# Autodesk Inventor assembly: Assembly
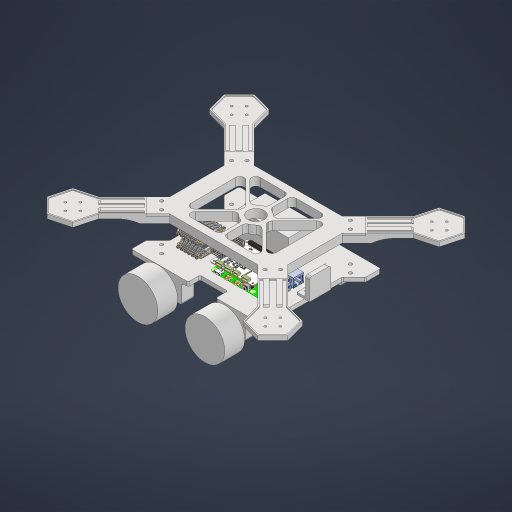
[picture p0: Inventor's stored thumbnail of the model, 512x512]
Saved by Autodesk Inventor 2023 (Build 270158000, 158)
## iProperties
Created: 2023-01-16
Part Number: Assembly
Document SubType Name: Assembly
Designer: Michael
Author: Michael
## Documents named in this file (12)
- D:\IDEs\Autodesk\SDP\Assembly.iam
- D:\IDEs\Autodesk\SDP\Base.ipt
- Electronics Panel.ipt
- D:\IDEs\Autodesk\SDP\navio2\NAVIO2.ipt
- D:\IDEs\Autodesk\SDP\raspberry-pi-4-model-b\Raspberry Pi 4 Model B.ipt
- D:\IDEs\Autodesk\SDP\tattu-4s-6750mah-lipo-battery\Tattu_4S_6750mAh_25C\Tattu_4S_6750mAh_25C.ipt
- D:\IDEs\Autodesk\SDP\LiPo.ipt
- D:\IDEs\Autodesk\SDP\ESC F45A\F45A.ipt
- D:\IDEs\Autodesk\SDP\Arm.ipt
- D:\IDEs\Autodesk\SDP\Top.ipt
- D:\IDEs\Autodesk\SDP\Camera Mount.ipt
- D:\IDEs\Autodesk\SDP\Mecanum Wheel.ipt
## Components (15 placed, 10 different names)
1. Electronics Panel:1 — Mate:25, Mate:26, Mate:33, Mate:34, Mate:35, Mate:36, Flush:5, Mate:39, Mate:40, Mate:41, Mate:42, Mate:43, Mate:44
2. NAVIO2:1 — Mate:5, Flush:1, Flush:2
3. Raspberry Pi 4 Model B:1 — Mate:5, Flush:1, Flush:2, Mate:25
4. Tattu_4S_6750mAh_25C:1 — Mate:40
5. LiPo:1 — Mate:39
6. F45A:1 — Mate:12, Flush:3, Flush:4, Mate:26, Mate:41, Mate:42, Flush:6
7. F45A:2 — Mate:12, Flush:3, Flush:4, Flush:6
8. Arm:2
9. Arm:3
10. Arm:4 — Mate:30, Mate:31, Mate:32
11. Arm:5
12. Top:1 — Mate:30, Mate:31, Mate:32, Mate:33, Flush:5
13. Camera Mount:1 — Mate:34, Mate:35, Mate:36
14. Mecanum Wheel:1 — Mate:43
15. Mecanum Wheel:2 — Mate:44
## Relationships (23: Mate 17, Flush 6)
- Mate:5 (10.16 mm): NAVIO2:1 ↔ Raspberry Pi 4 Model B:1
- Flush:1: NAVIO2:1 ↔ Raspberry Pi 4 Model B:1
- Flush:2: NAVIO2:1 ↔ Raspberry Pi 4 Model B:1
- Mate:12 (12.7 mm): F45A:1 ↔ F45A:2
- Flush:3: F45A:1 ↔ F45A:2
- Flush:4: F45A:1 ↔ F45A:2
- Mate:25: Electronics Panel:1 ↔ Raspberry Pi 4 Model B:1
- Mate:26: Electronics Panel:1 ↔ F45A:1
- Mate:30: Arm:4 ↔ Top:1
- Mate:31: Arm:4 ↔ Top:1
- Mate:32: Arm:4 ↔ Top:1
- Mate:33 (44.45 mm): Electronics Panel:1 ↔ Top:1
- Mate:34: Electronics Panel:1 ↔ Camera Mount:1
- Mate:35: Electronics Panel:1 ↔ Camera Mount:1
- Mate:36: Electronics Panel:1 ↔ Camera Mount:1
- Flush:5: Electronics Panel:1 ↔ Top:1
- Mate:39: Electronics Panel:1 ↔ LiPo:1
- Mate:40: Electronics Panel:1 ↔ Tattu_4S_6750mAh_25C:1
- Mate:41: Electronics Panel:1 ↔ F45A:1
- Mate:42: Electronics Panel:1 ↔ F45A:1
- Flush:6: F45A:1 ↔ F45A:2
- Mate:43 (12.7 mm): Electronics Panel:1 ↔ Mecanum Wheel:1
- Mate:44 (12.7 mm): Electronics Panel:1 ↔ Mecanum Wheel:2
